# Autodesk Inventor assembly: first_floor2
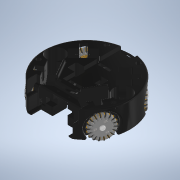
[picture p0: Inventor's stored thumbnail of the model, 180x180]
Saved by Autodesk Inventor 2020.4 (Build 244396000, 396)
## iProperties
Created: 2021-05-09
Part Number: first_floor2
Document SubType Name: Assembly
Designer: Acer
Author: Acer
## Documents named in this file (8)
- C:\Users\Acer\Documents\MATLAB\Doutorado\CAD\Inventor\first_floor\first_floor2.iam
- C:\Users\Acer\Documents\MATLAB\Doutorado\CAD\Inventor\first_floor\Base_RoboCIn.ipt
- C:\Users\Acer\Documents\MATLAB\Doutorado\CAD\Inventor\first_floor\dribbler-3-gears\Dribbler-3-gears-new.iam
- C:\Users\Acer\Documents\MATLAB\Doutorado\CAD\Inventor\first_floor\Components\M5Nut_Special.ipt
- C:\Users\Acer\Documents\MATLAB\Doutorado\CAD\Inventor\first_floor\Motor\MaxonEC45-50W-MILE-Machined-with-gear.iam
- C:\Users\Acer\Documents\MATLAB\Doutorado\CAD\Inventor\first_floor\Wheel\RoboCinWheel.iam
- C:\Users\Acer\Documents\MATLAB\Doutorado\CAD\Inventor\first_floor\Components\Battery4S.ipt
- C:\Users\Acer\Documents\MATLAB\Doutorado\CAD\Inventor\first_floor\Components\Capacitor.ipt
## Components (17 placed, 7 different names)
1. Base_RoboCIn:1 — Mate:1, Mate:2, Mate:3, Mate:4, Mate:5, Mate:6, Mate:7, Mate:8, Mate:9, Mate:10, Mate:11, Mate:12, Mate:13, Mate:14, Mate:15, Mate:16, Mate:17, Mate:18, Mate:19, Mate:20, Mate:21, Mate:22, Mate:23, Mate:24, Mate:25, Mate:26, Mate:27, Mate:28, Mate:29, Mate:30, Mate:31, Mate:32, Mate:33, Mate:34, Mate:35, Mate:38, Mate:39, Mate:40, Mate:41, Mate:42, Mate:43, Mate:44
2. Dribbler-3-gears-new:1 [sub-assembly] — Mate:1, Mate:2
3. M5Nut_Special:1 — Mate:3, Mate:4, Mate:5
4. M5Nut_Special:2 — Mate:12, Mate:13, Mate:14
5. M5Nut_Special:3 — Mate:9, Mate:10, Mate:11
6. M5Nut_Special:4 — Mate:6, Mate:7, Mate:8
7. MG-MaxonEC45-50W-MILE:1 [sub-assembly] — Mate:15, Mate:16, Mate:17
8. MG-MaxonEC45-50W-MILE:2 [sub-assembly] — Mate:18, Mate:19, Mate:20, Mate:21
9. MG-MaxonEC45-50W-MILE:3 [sub-assembly] — Mate:22, Mate:23, Mate:24
10. MG-MaxonEC45-50W-MILE:4 [sub-assembly] — Mate:25, Mate:26, Mate:27
11. RoboCinWheel:1 [sub-assembly] — Mate:28, Mate:29
12. RoboCinWheel:2 [sub-assembly] — Mate:30, Mate:31
13. RoboCinWheel:3 [sub-assembly] — Mate:34, Mate:35
14. RoboCinWheel:4 [sub-assembly] — Mate:32, Mate:33
15. Battery4S:1 — Mate:38, Mate:39, Mate:40
16. Capacitor:1 — Mate:43, Mate:44
17. Capacitor:2 — Mate:41, Mate:42
## Relationships (42: Mate 42)
- Mate:1: Base_RoboCIn:1 ↔ Dribbler-3-gears-new:1
- Mate:2 (0.25 mm): Base_RoboCIn:1 ↔ Dribbler-3-gears-new:1
- Mate:3: Base_RoboCIn:1 ↔ M5Nut_Special:1
- Mate:4: Base_RoboCIn:1 ↔ M5Nut_Special:1
- Mate:5: Base_RoboCIn:1 ↔ M5Nut_Special:1
- Mate:6: Base_RoboCIn:1 ↔ M5Nut_Special:4
- Mate:7: Base_RoboCIn:1 ↔ M5Nut_Special:4
- Mate:8: Base_RoboCIn:1 ↔ M5Nut_Special:4
- Mate:9: Base_RoboCIn:1 ↔ M5Nut_Special:3
- Mate:10: Base_RoboCIn:1 ↔ M5Nut_Special:3
- Mate:11: Base_RoboCIn:1 ↔ M5Nut_Special:3
- Mate:12: Base_RoboCIn:1 ↔ M5Nut_Special:2
- Mate:13: Base_RoboCIn:1 ↔ M5Nut_Special:2
- Mate:14: Base_RoboCIn:1 ↔ M5Nut_Special:2
- Mate:15: Base_RoboCIn:1 ↔ MG-MaxonEC45-50W-MILE:1
- Mate:16: Base_RoboCIn:1 ↔ MG-MaxonEC45-50W-MILE:1
- Mate:17: Base_RoboCIn:1 ↔ MG-MaxonEC45-50W-MILE:1
- Mate:18: Base_RoboCIn:1 ↔ MG-MaxonEC45-50W-MILE:2
- Mate:19: Base_RoboCIn:1 ↔ MG-MaxonEC45-50W-MILE:2
- Mate:20: Base_RoboCIn:1 ↔ MG-MaxonEC45-50W-MILE:2
- Mate:21: Base_RoboCIn:1 ↔ MG-MaxonEC45-50W-MILE:2
- Mate:22: Base_RoboCIn:1 ↔ MG-MaxonEC45-50W-MILE:3
- Mate:23: Base_RoboCIn:1 ↔ MG-MaxonEC45-50W-MILE:3
- Mate:24: Base_RoboCIn:1 ↔ MG-MaxonEC45-50W-MILE:3
- Mate:25: Base_RoboCIn:1 ↔ MG-MaxonEC45-50W-MILE:4
- Mate:26: Base_RoboCIn:1 ↔ MG-MaxonEC45-50W-MILE:4
- Mate:27: Base_RoboCIn:1 ↔ MG-MaxonEC45-50W-MILE:4
- Mate:28: Base_RoboCIn:1 ↔ RoboCinWheel:1
- Mate:29 (1 mm): Base_RoboCIn:1 ↔ RoboCinWheel:1
- Mate:30: Base_RoboCIn:1 ↔ RoboCinWheel:2
- Mate:31 (1 mm): Base_RoboCIn:1 ↔ RoboCinWheel:2
- Mate:32: Base_RoboCIn:1 ↔ RoboCinWheel:4
- Mate:33 (1 mm): Base_RoboCIn:1 ↔ RoboCinWheel:4
- Mate:34: Base_RoboCIn:1 ↔ RoboCinWheel:3
- Mate:35 (1 mm): Base_RoboCIn:1 ↔ RoboCinWheel:3
- Mate:38: Base_RoboCIn:1 ↔ Battery4S:1
- Mate:39 (1 mm): Base_RoboCIn:1 ↔ Battery4S:1
- Mate:40 (1 mm): Base_RoboCIn:1 ↔ Battery4S:1
- Mate:41: Base_RoboCIn:1 ↔ Capacitor:2
- Mate:42: Base_RoboCIn:1 ↔ Capacitor:2
- Mate:43: Base_RoboCIn:1 ↔ Capacitor:1
- Mate:44: Base_RoboCIn:1 ↔ Capacitor:1
